# Autodesk Inventor assembly: HACKberry_v1_for_print_Hand_withCase
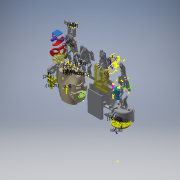
[picture p0: Inventor's stored thumbnail of the model, 180x180]
Saved by Autodesk Inventor 2016 (Build 200138000, 138)
## iProperties
Created: 2015-02-09
Part Number: HACKberry_v1_for_print_Hand_withCase
Document SubType Name: Assembly
Designer: Yamaura
Author: Yamaura
## Documents named in this file (13)
- C:\Users\Yamaura\Documents\GitHub\HACKberry\HACKberry-hardware\3D\Inventor\HACKberry_v1_for_print_Hand_withCase.iam
- C:\Users\Yamaura\Documents\GitHub\HACKberry\HACKberry-hardware\3D\Inventor\Parts\HbPalmBase03.ipt
- C:\Users\Yamaura\Documents\GitHub\HACKberry\HACKberry-hardware\3D\Inventor\Parts\HbBackCover02.ipt
- C:\Users\Yamaura\Documents\GitHub\HACKberry\HACKberry-hardware\3D\Inventor\Parts\HbBatteryCaseHolder01.ipt
- C:\Users\Yamaura\Documents\GitHub\HACKberry\HACKberry-hardware\3D\Inventor\Parts\HbThumbLockButton01.ipt
- C:\Users\Yamaura\Documents\GitHub\HACKberry\HACKberry-hardware\3D\Inventor\Parts\HbThumbJointHolder01.ipt
- C:\Users\Yamaura\Documents\GitHub\HACKberry\HACKberry-hardware\3D\Inventor\Parts\HbThumbProximalPhalanx02.ipt
- C:\Users\Yamaura\Documents\GitHub\HACKberry\HACKberry-hardware\3D\Inventor\Parts\HbPrintCaseForSLS02.ipt
- C:\Users\Yamaura\Documents\GitHub\HACKberry\HACKberry-hardware\3D\Inventor\Parts\HACKberry_v1_for_print_Hand_withCaseB.iam
- C:\Users\Yamaura\Documents\GitHub\HACKberry\HACKberry-hardware\3D\Inventor\Parts\HACKberry_v1_for_print_Hand_withCaseC.iam
- C:\Users\Yamaura\Documents\GitHub\HACKberry\HACKberry-hardware\3D\Inventor\Parts\HACKberry_v1_for_print_Hand_withCaseA.iam
- C:\Users\Yamaura\Documents\GitHub\HACKberry\HACKberry-hardware\3D\Inventor\Parts\HACKberry_v1_for_print_Hand_withCaseD.iam
- C:\Users\Yamaura\Documents\GitHub\HACKberry\HACKberry-hardware\3D\Inventor\Parts\HACKberry_v1_for_print_Hand_withCaseE.iam
## Components (12 placed, 12 different names)
1. HbPalmBase03:1
2. HbBackCover02:1 — メイト:30
3. HbBatteryCaseHolder01:1
4. HbThumbLockButton01:1
5. HbThumbJointHolder01:1
6. HbThumbProximalPhalanx02:1
7. HbPrintCaseForSLS02:1 — フラッシュ:3, フラッシュ:4
8. HACKberry_v1_for_print_Hand_withCaseA:1 [sub-assembly]
9. HACKberry_v1_for_print_Hand_withCaseB:1 [sub-assembly]
10. HACKberry_v1_for_print_Hand_withCaseC:1 [sub-assembly]
11. HACKberry_v1_for_print_Hand_withCaseD:1 [sub-assembly]
12. HACKberry_v1_for_print_Hand_withCaseE:1 [sub-assembly]
## Relationships (4: Flush 3, Mate 1)
- メイト:30 [Mate]: HbBackCover02:1
- フラッシュ:2 [Flush] (50 mm)
- フラッシュ:3 [Flush]: HbPrintCaseForSLS02:1
- フラッシュ:4 [Flush]: HbPrintCaseForSLS02:1
